# Autodesk Inventor assembly: Rigid Box
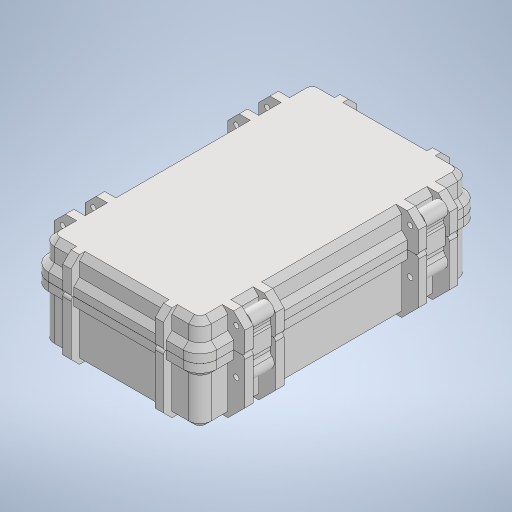
[picture p0: Inventor's stored thumbnail of the model, 512x512]
Saved by Autodesk Inventor 2023.4 (Build 274418000, 418)
## iProperties
Created: 2024-07-02
Part Number: Rigid Box
Document SubType Name: Assembly
Designer: Nathan Cai
Author: Nathan Cai
## Documents named in this file (4)
- E:\Documents\Inventor\Misc\Rigid Box\Rigid Box.iam
- E:\Documents\Inventor\Misc\Rigid Box\Shell.ipt
- E:\Documents\Inventor\Misc\Rigid Box\Shell - Low.ipt
- E:\Documents\Inventor\Misc\Rigid Box\Hinge.ipt
## Components (4 placed, 3 different names)
1. Shell:1 — Flush:1, Mate:2, Mate:4, Mate:7
2. Shell - Low:1 — Flush:1, Mate:1, Mate:3, Mate:5, Mate:6
3. Hinge:1 — Mate:1, Mate:2, Mate:3, Mate:4
4. Hinge:2 — Mate:5, Mate:6, Mate:7
## Relationships (8: Mate 7, Flush 1)
- Flush:1: Shell:1 ↔ Shell - Low:1
- Mate:1: Shell - Low:1 ↔ Hinge:1
- Mate:2: Shell:1 ↔ Hinge:1
- Mate:3: Shell - Low:1 ↔ Hinge:1
- Mate:4: Shell:1 ↔ Hinge:1
- Mate:5: Shell - Low:1 ↔ Hinge:2
- Mate:6: Shell - Low:1 ↔ Hinge:2
- Mate:7: Shell:1 ↔ Hinge:2
